# Autodesk Inventor assembly: 000.007 - Куб типа Ш (красный)
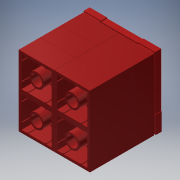
[picture p0: Inventor's stored thumbnail of the model, 180x180]
Saved by Autodesk Inventor 2019 (Build 230136000, 136)
## iProperties
Created: 2020-02-29
Part Number: 000.007 - Куб типа Ш (красный)
Material: Типовые
Document SubType Name: Assembly
Designer: Петров Иван
Author: Петров Иван
## Documents named in this file (3)
- E:\IVAN\Ivan_desktop\GitHub\Manipulation_IRS\hardware\000.007 - Куб типа Ш (красный).iam
- E:\IVAN\Ivan_desktop\GitHub\Manipulation_IRS\hardware\components\modular-lego-brick-standard-1.snapshot.7\Brick standard 4x2.ipt
- E:\IVAN\Ivan_desktop\GitHub\Manipulation_IRS\hardware\components\modular-lego-brick-standard-1.snapshot.7\1x4 flat RED.ipt
## Components (10 placed, 2 different names)
1. 1x4 flat RED:1 — Заподлицо:7, Заподлицо:8, Заподлицо:9
2. 1x4 flat RED:2 — Заподлицо:10, Заподлицо:11, Заподлицо:12
3. 1x4 flat RED:3 — Заподлицо:3, Совмещение:2, Заподлицо:4, Заподлицо:7, Заподлицо:9, Заподлицо:10, Заподлицо:11
4. 1x4 flat RED:4 — Совмещение:3, Заподлицо:5, Заподлицо:6, Заподлицо:8, Заподлицо:12
5. Brick standard 4x2:2 — Совмещение:1, Заподлицо:1, Заподлицо:2
6. Brick standard 4x2:1 — Совмещение:1, Заподлицо:1, Заподлицо:2
7. Brick standard 4x2:3
8. Brick standard 4x2:4
9. Brick standard 4x2:5 — Заподлицо:4
10. Brick standard 4x2:6 — Заподлицо:3, Совмещение:2, Совмещение:3, Заподлицо:5, Заподлицо:6
## Component patterns: (3 elements, first: Brick standard 4x2:2 + Brick standard 4x2:1)
## Relationships (15: Flush 12, Mate 3)
- Совмещение:1 [Mate]: Brick standard 4x2:2 ↔ Brick standard 4x2:1
- Заподлицо:1 [Flush]: Brick standard 4x2:2 ↔ Brick standard 4x2:1
- Заподлицо:2 [Flush]: Brick standard 4x2:2 ↔ Brick standard 4x2:1
- Заподлицо:3 [Flush]: 1x4 flat RED:3 ↔ Brick standard 4x2:6
- Совмещение:2 [Mate]: 1x4 flat RED:3 ↔ Brick standard 4x2:6
- Заподлицо:4 [Flush]: 1x4 flat RED:3 ↔ Brick standard 4x2:5
- Совмещение:3 [Mate]: 1x4 flat RED:4 ↔ Brick standard 4x2:6
- Заподлицо:5 [Flush]: 1x4 flat RED:4 ↔ Brick standard 4x2:6
- Заподлицо:6 [Flush]: 1x4 flat RED:4 ↔ Brick standard 4x2:6
- Заподлицо:7 [Flush]: 1x4 flat RED:1 ↔ 1x4 flat RED:3
- Заподлицо:8 [Flush]: 1x4 flat RED:1 ↔ 1x4 flat RED:4
- Заподлицо:9 [Flush]: 1x4 flat RED:1 ↔ 1x4 flat RED:3
- Заподлицо:10 [Flush]: 1x4 flat RED:2 ↔ 1x4 flat RED:3
- Заподлицо:11 [Flush]: 1x4 flat RED:2 ↔ 1x4 flat RED:3
- Заподлицо:12 [Flush]: 1x4 flat RED:2 ↔ 1x4 flat RED:4
